# Autodesk Inventor assembly: PCB
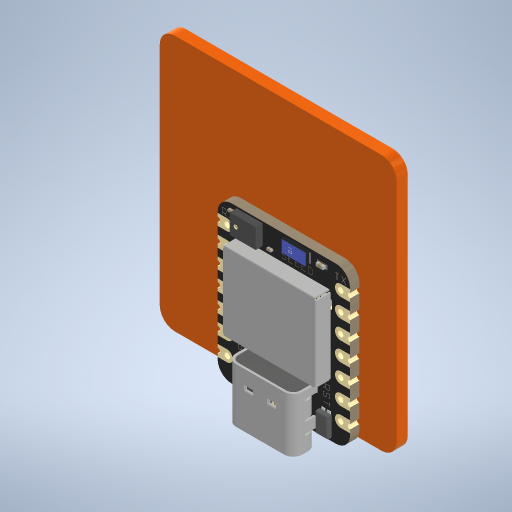
[picture p0: Inventor's stored thumbnail of the model, 512x512]
Saved by Autodesk Inventor 2024.3 (Build 283343000, 343)
## iProperties
Created: 2024-11-30
Part Number: PCB
Document SubType Name: Assembly
Designer: ASUS TUF
Author: ASUS TUF
## Documents named in this file (3)
- C:\Users\ASUS TUF\Documents\Inventor\ParkinsonDetection\PCB.iam
- C:\Users\ASUS TUF\Documents\Inventor\ParkinsonDetection\PCB-V1.ipt
- C:\Users\ASUS TUF\Documents\Inventor\ParkinsonDetection\XIAO-nRF52840 v15\XIAO-nRF52840 v15\XIAO-nRF52840 v15.iam
## Components (2 placed, 2 different names)
1. PCB-V1:1 — Mate:1, Flush:1, Flush:2
2. XIAO-nRF52840 v15:1 [sub-assembly] — Mate:1, Flush:1, Flush:2
## Relationships (3: Flush 2, Mate 1)
- Mate:1 (3 mm): PCB-V1:1 ↔ XIAO-nRF52840 v15:1
- Flush:1 (2 mm): PCB-V1:1 ↔ XIAO-nRF52840 v15:1
- Flush:2 (2 mm): PCB-V1:1 ↔ XIAO-nRF52840 v15:1
